# Autodesk Inventor assembly: Instrumentation Panel
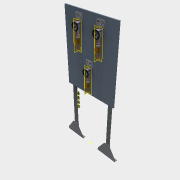
[picture p0: Inventor's stored thumbnail of the model, 180x180]
Saved by Autodesk Inventor 2019.1 (Build 231200000, 200)
## iProperties
Created: 2009-08-11
Part Number: Instrumentation Panel
Document SubType Name: Assembly
Designer: Demir Ali
Mass: 79043.7 g
Surface Area: 59039.2 cm^2
Volume: 58957.2 cm^3
Density: 1.3407 g/cm^3
Description: Instrumentation Panel
Stock Number: NA
_SolveAssemblyDoc: Frame Generator Solve Assembly
_Version: 15.0.0
Author: Demir Ali
Title: Manufactured Part
Revision Number: A
## Documents named in this file (10)
- C:\Vault Workspace\Process Equipment\Workspace\Options\Instrumentation Panel.iam
- C:\Vault Workspace\Process Equipment\Workspace\Components\Instrumentation_Frame_SK.ipt
- C:\Vault Workspace\Process Equipment\Workspace\Framework\Instrumentation Panel Board.ipt
- C:\Vault Workspace\Process Equipment\Workspace\Supplier Content\Pressure Gauge\PI-101.iam
- C:\Vault Workspace\Process Equipment\Workspace\Supplier Content\Pressure Gauge\PI-101_Instrument Name Plate.ipt
- C:\Vault Workspace\Process Equipment\Workspace\Supplier Content\Pressure Gauge\PI-102_Instrument Name Plate.ipt
- C:\Vault Workspace\Process Equipment\Workspace\Supplier Content\Pressure Gauge\PI-103_Instrument Name Plate.ipt
- C:\Vault Workspace\Process Equipment\Workspace\Framework\Instrumentation Panel\Frame\PI-Panel-Frame.iam
- C:\Vault Workspace\Process Equipment\Workspace\Supplier Content\P2348-S1-Unistrut.ipt
- C:\Vault Workspace\Process Equipment\Workspace\Supplier Content\Pipe Clamp - 25.ipt
## Components (15 placed, 9 different names)
1. Instrumentation_Frame_SK:1 — Angle:1, Angle:2, Mate:10, Mate:9
2. Instrumentation Panel Board:1 — Mate:1, Mate:2, Mate:3, Mate:7, Mate:8
3. PI-101_Instrument Name Plate:1 — Mate:3, Flush:1, Flush:2, Flush:3, Flush:4, Flush:6, Flush:11
4. PI-102_Instrument Name Plate:1 — Flush:3, Flush:6, Flush:10
5. PI-103_Instrument Name Plate:1 — Flush:4, Flush:11
6. PI-Panel-Frame:1 [sub-assembly] — Mate:4, Mate:5, Mate:6, Mate:11
7. PI-101:3 [sub-assembly] — Mate:7, Mate:8, Angle:2
8. PI-101:1 [sub-assembly] — Mate:1, Mate:2, Angle:1, Flush:1, Flush:2
9. PI-101:2 [sub-assembly] — Flush:10
10. P2348-S1-Unistrut:1 — Mate:4, Mate:5, Mate:6
11. P2348-S1-Unistrut:2
12. Pipe Clamp - 25:1 — Mate:10, Mate:11, Mate:9
13. Pipe Clamp - 25:2
14. Pipe Clamp - 25:3
15. Pipe Clamp - 25:4
## Component patterns: (2 elements, first: PI-101:1), (2 elements, first: P2348-S1-Unistrut:1), (4 elements, first: Pipe Clamp - 25:1)
## Relationships (21: Mate 11, Flush 8, Angle 2)
- Mate:1: Instrumentation Panel Board:1 ↔ PI-101:1
- Mate:2: Instrumentation Panel Board:1 ↔ PI-101:1
- Angle:1 (0 deg): Instrumentation_Frame_SK:1 ↔ PI-101:1
- Mate:3: Instrumentation Panel Board:1 ↔ PI-101_Instrument Name Plate:1
- Flush:1: PI-101_Instrument Name Plate:1 ↔ PI-101:1
- Flush:2 (-100 mm): PI-101_Instrument Name Plate:1 ↔ PI-101:1
- Flush:3: PI-101_Instrument Name Plate:1 ↔ PI-102_Instrument Name Plate:1
- Flush:4: PI-101_Instrument Name Plate:1 ↔ PI-103_Instrument Name Plate:1
- Flush:6: PI-101_Instrument Name Plate:1 ↔ PI-102_Instrument Name Plate:1
- [Flush]: PI-103_Instrument Name Plate:1 ↔ PI-101:3
- Flush:10: PI-102_Instrument Name Plate:1 ↔ PI-101:2
- Flush:11 (-500 mm): PI-101_Instrument Name Plate:1 ↔ PI-103_Instrument Name Plate:1
- Mate:4: PI-Panel-Frame:1 ↔ P2348-S1-Unistrut:1
- Mate:5: PI-Panel-Frame:1 ↔ P2348-S1-Unistrut:1
- Mate:6: PI-Panel-Frame:1 ↔ P2348-S1-Unistrut:1
- Mate:7: Instrumentation Panel Board:1 ↔ PI-101:3
- Mate:8: Instrumentation Panel Board:1 ↔ PI-101:3
- Angle:2 (0 deg): Instrumentation_Frame_SK:1 ↔ PI-101:3
- Mate:10 (20 mm): Instrumentation_Frame_SK:1 ↔ Pipe Clamp - 25:1
- Mate:11 (-20 mm): PI-Panel-Frame:1 ↔ Pipe Clamp - 25:1
- Mate:9 (692 mm): Instrumentation_Frame_SK:1 ↔ Pipe Clamp - 25:1
